# Autodesk Inventor assembly: Assembly5
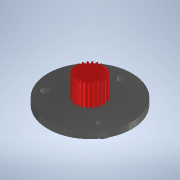
[picture p0: Inventor's stored thumbnail of the model, 180x180]
Saved by Autodesk Inventor 2022 (Build 260153000, 153)
## iProperties
Created: 2022-04-03
Part Number: Assembly5
Document SubType Name: Assembly
Designer: Mlees
Author: Mlees
## Documents named in this file (3)
- C:\Users\Mlees\Desktop\504Engineering\Project_0000\Designs\Design_1\Created_Parts\Assembly5.iam
- C:\Users\Mlees\Desktop\504Engineering\Project_0000\Designs\Design_1\Created_Parts\Plamet_Carrier.ipt
- C:\Users\Mlees\Desktop\504Engineering\Project_0000\Designs\Design_1\Created_Parts\24_Teeth_Sun_Gear_mod.ipt
## Components (2 placed, 2 different names)
1. Plamet_Carrier:1 — Rigid:1
2. 24_Teeth_Sun_Gear_mod:1 — Rigid:1
## Relationships (1: WeldJoint 1)
- Rigid:1 [WeldJoint]: Plamet_Carrier:1 ↔ 24_Teeth_Sun_Gear_mod:1
